# Autodesk Inventor assembly: Assembly1
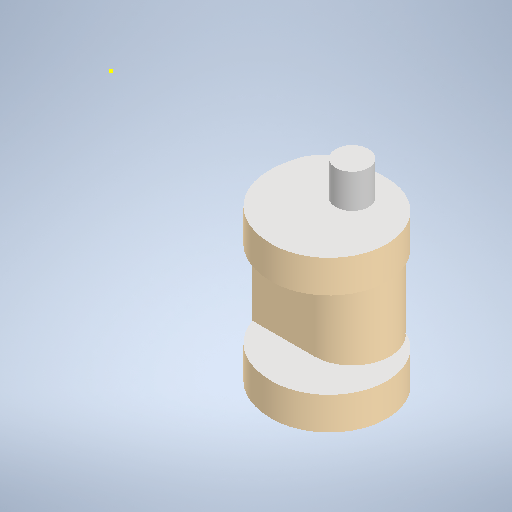
[picture p0: Inventor's stored thumbnail of the model, 512x512]
Saved by Autodesk Inventor 2025.1 (Build 291241000, 241)
## iProperties
Created: 2025-02-27
Part Number: Assembly1
Document SubType Name: Assembly
Designer: santiago
Author: santiago
## Documents named in this file (3)
- C:\Users\santiago\Documents\Tesis\3d models\scaled\CUSTOM\Assembly1.iam
- C:\Users\santiago\Documents\Tesis\3d models\scaled\cam.ipt
- C:\Users\santiago\Documents\Tesis\3d models\scaled\axis.ipt
## Components (3 placed, 2 different names)
1. cam:1 — Mate:1, Mate:2
2. axis:1 — Mate:1
3. axis:2 — Mate:2
## Relationships (2: Mate 2)
- Mate:1: cam:1 ↔ axis:1
- Mate:2: cam:1 ↔ axis:2
